# Autodesk Inventor assembly: Kocepcja
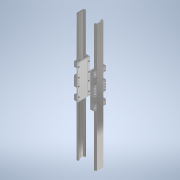
[picture p0: Inventor's stored thumbnail of the model, 180x180]
Saved by Autodesk Inventor 2020 (Build 240168000, 168)
## iProperties
Created: 2022-04-22
Part Number: Kocepcja
Document SubType Name: Assembly
Designer: mikoma
Author: mikoma
## Documents named in this file (3)
- D:\KONIECTEGOKOŁCHOZU\MGR\model\Workspaces\Obszar roboczy\Assembly_v3\Kocepcja.iam
- D:\KONIECTEGOKOŁCHOZU\MGR\model\Workspaces\Obszar roboczy\Assembly_v1\X\WS_10_40_X.ipt
- D:\KONIECTEGOKOŁCHOZU\MGR\model\Workspaces\Obszar roboczy\Zawartość\Igus\WW_10_40_10_2.ipt
## Components (6 placed, 2 different names)
1. WW_10_40_10_2:1 — Zestawiające:5, Zestawiające:6, Zestawiające:9, Równoległe:3
2. WW_10_40_10_2:2 — Zestawiające:10, Zestawiające:11, Zestawiające:14
3. WW_10_40_10_2:3 — Zestawiające:7, Zestawiające:8, Zestawiające:9
4. WW_10_40_10_2:4 — Zestawiające:12, Zestawiające:13, Zestawiające:14, Równoległe:3
5. WS_10_40_X:1 — Zestawiające:1, Zestawiające:2, Zestawiające:3, Równoległe:1, Kątowe:1, Równoległe:2, Zestawiające:4, Zestawiające:5, Zestawiające:6, Zestawiające:7, Zestawiające:8
6. WS_10_40_X:2 — Równoległe:1, Kątowe:1, Równoległe:2, Zestawiające:4, Zestawiające:10, Zestawiające:11, Zestawiające:12, Zestawiające:13
## Relationships (18: Mate 14, Flush 3, Angle 1)
- Zestawiające:1 [Mate]: WS_10_40_X:1
- Zestawiające:2 [Mate]: WS_10_40_X:1
- Zestawiające:3 [Mate]: WS_10_40_X:1
- Równoległe:1 [Flush]: WS_10_40_X:1 ↔ WS_10_40_X:2
- Kątowe:1 [Angle] (180 deg): WS_10_40_X:1 ↔ WS_10_40_X:2
- Równoległe:2 [Flush]: WS_10_40_X:1 ↔ WS_10_40_X:2
- Zestawiające:4 [Mate] (-120 mm): WS_10_40_X:1 ↔ WS_10_40_X:2
- Zestawiające:5 [Mate]: WW_10_40_10_2:1 ↔ WS_10_40_X:1
- Zestawiające:6 [Mate]: WW_10_40_10_2:1 ↔ WS_10_40_X:1
- Zestawiające:7 [Mate]: WW_10_40_10_2:3 ↔ WS_10_40_X:1
- Zestawiające:8 [Mate]: WW_10_40_10_2:3 ↔ WS_10_40_X:1
- Zestawiające:9 [Mate]: WW_10_40_10_2:1 ↔ WW_10_40_10_2:3
- Zestawiające:10 [Mate]: WW_10_40_10_2:2 ↔ WS_10_40_X:2
- Zestawiające:11 [Mate]: WW_10_40_10_2:2 ↔ WS_10_40_X:2
- Zestawiające:12 [Mate]: WW_10_40_10_2:4 ↔ WS_10_40_X:2
- Zestawiające:13 [Mate]: WW_10_40_10_2:4 ↔ WS_10_40_X:2
- Zestawiające:14 [Mate]: WW_10_40_10_2:2 ↔ WW_10_40_10_2:4
- Równoległe:3 [Flush]: WW_10_40_10_2:1 ↔ WW_10_40_10_2:4
